# Autodesk Inventor assembly: Telescope
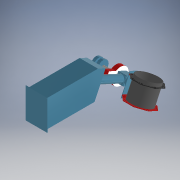
[picture p0: Inventor's stored thumbnail of the model, 180x180]
Saved by Autodesk Inventor 2022 (Build 260153000, 153)
## iProperties
Created: 2021-04-24
Part Number: Telescope
Document SubType Name: Assembly
Designer: Mick Veldhuis
Author: Mick Veldhuis
## Documents named in this file (4)
- C:\Users\Mick Veldhuis\Desktop\bsc-project\inventor\observatory\Telescope.iam
- C:\Users\Mick Veldhuis\Desktop\bsc-project\inventor\observatory\TelescopeMount.iam
- TelescopeMount.iam
- C:\Users\Mick Veldhuis\Desktop\bsc-project\inventor\observatory\TelescopeOptics.iam
## Components (2 placed, 2 different names)
1. TelescopeMount:1 [sub-assembly] — Insert:1, Angle:1
2. TelescopeOptics:1 [sub-assembly] — Insert:1, Angle:1
## Relationships (2: Insert 1, Angle 1)
- Insert:1 (8 mm): TelescopeMount:1 ↔ TelescopeOptics:1
- Angle:1 (0 deg): TelescopeMount:1 ↔ TelescopeOptics:1
